# Autodesk Inventor assembly: Leg_Right
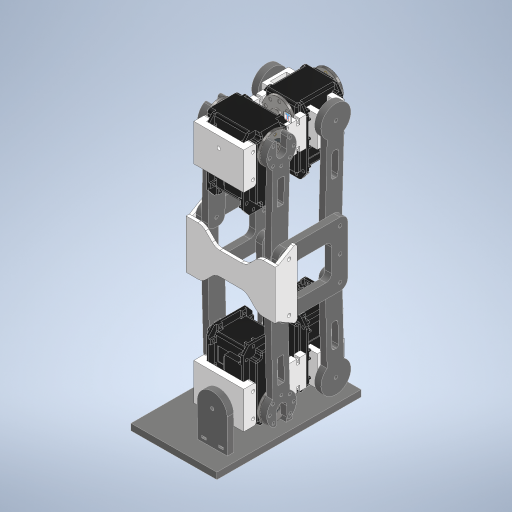
[picture p0: Inventor's stored thumbnail of the model, 512x512]
Saved by Autodesk Inventor 2024.3 (Build 283343000, 343)
## iProperties
Created: 2024-09-18
Part Number: Leg_Right
Document SubType Name: Assembly
Designer: 구지현
Author: 구지현
## Documents named in this file (20)
- C:\Users\구지현\Desktop\19th_intern_kdy_robot\부품\Lower_Body\Leg\Leg_Right.iam
- C:\Users\구지현\Documents\카카오톡 받은 파일\Hardware\ROBOTIS(Inventor 2024 ver.)\다이나믹셀\MX-64T+idle.ipt.iam
- C:\Users\구지현\Documents\카카오톡 받은 파일\Hardware\ROBOTIS(Inventor 2024 ver.)\다이나믹셀\MX-106T+idle.ipt.iam
- C:\Users\구지현\Documents\카카오톡 받은 파일\Hardware\ROBOTIS(Inventor 2024 ver.)\혼\64-106Horn.ipt
- C:\Users\구지현\Desktop\19th_intern_kdy_robot\부품\Lower_Body\Leg\Back_Ankle.ipt
- C:\Users\구지현\Desktop\19th_intern_kdy_robot\부품\Lower_Body\Leg\Foot_MIR.ipt
- C:\Users\구지현\Desktop\19th_intern_kdy_robot\부품\Lower_Body\Leg\Front_Ankle.ipt
- C:\Users\구지현\Desktop\19th_intern_kdy_robot\부품\Lower_Body\Leg\Knee.ipt
- C:\Users\구지현\Desktop\19th_intern_kdy_robot\부품\Lower_Body\Leg\Knee_Covers.ipt
- C:\Users\구지현\Desktop\19th_intern_kdy_robot\부품\Lower_Body\Leg\Leg_Connection_Parts_Back.ipt
- C:\Users\구지현\Desktop\19th_intern_kdy_robot\부품\Lower_Body\Leg\Leg_Connection_Parts_Front.ipt
- C:\Users\구지현\Desktop\19th_intern_kdy_robot\부품\Lower_Body\Leg\Leg_Foot_Connection_Parts.ipt
- C:\Users\구지현\Desktop\19th_intern_kdy_robot\부품\Lower_Body\Leg\Link_Fixation_Connector.ipt
- C:\Users\구지현\Desktop\19th_intern_kdy_robot\부품\Lower_Body\Leg\Link_Fixation_Connector_MIR.ipt
- Link_Fixation_Connector_left_left.ipt
- C:\Users\구지현\Desktop\19th_intern_kdy_robot\부품\Lower_Body\Leg\Link_Fixation_Connector_MIR_MIR.ipt
- C:\Users\구지현\Desktop\19th_intern_kdy_robot\부품\Lower_Body\Leg\Link_Fixation_Connector_MIR1.ipt
- C:\Users\구지현\Desktop\19th_intern_kdy_robot\부품\Lower_Body\Leg\Vertical_Fixation_Set.iam
- MX-106T+idle.ipt
- MX-64T+idle.ipt
## Components (32 placed, 16 different names)
1. MX-106T+idle.ipt:3 [sub-assembly] — 플러쉬:9, 각도:4, 플러쉬:10, 메이트:24, 메이트:25, 삽입:26, 삽입:27, 삽입:28, 삽입:29, 메이트:34, 메이트:35, 메이트:36
2. 64-106Horn:5 — 메이트:22, 메이트:23
3. MX-106T+idle.ipt:4 [sub-assembly] — 메이트:1, 메이트:2, 메이트:3, 메이트:6, 메이트:7, 메이트:8, 메이트:10, 메이트:11, 플러쉬:9, 각도:4, 플러쉬:10
4. 64-106Horn:6 — 메이트:12, 메이트:13
5. MX-64T+idle.ipt:3 [sub-assembly] — 플러쉬:13, 플러쉬:14, 삽입:30, 삽입:31, 삽입:32, 삽입:33, 삽입:34, 메이트:26, 메이트:27, 메이트:28, 메이트:30, 메이트:31, 메이트:32
6. 64-106Horn:7
7. MX-64T+idle.ipt:4 [sub-assembly] — 삽입:12, 메이트:9, 메이트:14, 메이트:15, 메이트:16, 메이트:18, 메이트:19, 메이트:20, 플러쉬:13, 플러쉬:14
8. 64-106Horn:8 — 삽입:10
9. Back_Ankle:1 — 삽입:10, 플러쉬:1, 각도:1, 삽입:14
10. Foot_MIR:1 — 삽입:13, 삽입:14
11. Front_Ankle:1 — 삽입:11, 플러쉬:1, 각도:1, 삽입:13
12. Knee:1 — 삽입:15, 삽입:18, 플러쉬:6, 플러쉬:7, 삽입:20, 삽입:21, 삽입:25, 삽입:36
13. Knee_Covers:1 — 삽입:20, 삽입:21, 삽입:22, 삽입:23
14. Leg_Connection_Parts_Front:1 — 메이트:12, 메이트:13, 플러쉬:2, 플러쉬:3, 삽입:15, 플러쉬:4, 각도:2
15. Leg_Foot_Connection_Parts:1 — 메이트:6, 메이트:7, 메이트:8, 삽입:11, 플러쉬:18
16. Link_Fixation_Connector_left_left:1 — 메이트:14, 메이트:15, 메이트:16, 메이트:17
17. Vertical_Fixation_Set:1 [sub-assembly] — 메이트:1, 메이트:2, 메이트:3, 삽입:12, 메이트:9
18. Leg_Connection_Parts_Front:2 — 메이트:10, 메이트:11, 플러쉬:2, 플러쉬:3, 삽입:17, 플러쉬:5, 각도:3
19. Link_Fixation_Connector_MIR1:2
20. Leg_Connection_Parts_Back:4 — 플러쉬:4, 각도:2, 삽입:18, 플러쉬:8, 메이트:21
21. Leg_Connection_Parts_Back:5 — 플러쉬:5, 각도:3, 삽입:19, 플러쉬:8, 메이트:17
22. Knee:2 — 삽입:17, 플러쉬:6, 플러쉬:7, 삽입:19, 삽입:22, 삽입:23, 삽입:24, 삽입:35
23. Link_Fixation_Connector:2 — 메이트:18, 메이트:19, 메이트:20, 메이트:21
24. Link_Fixation_Connector_MIR1:4 — 메이트:26, 메이트:27, 메이트:28, 메이트:29
25. Link_Fixation_Connector:3
26. Leg_Connection_Parts_Front:3 — 메이트:24, 메이트:25, 플러쉬:11, 플러쉬:12, 삽입:24, 플러쉬:15, 각도:5
27. Leg_Connection_Parts_Front:4 — 메이트:22, 메이트:23, 플러쉬:11, 플러쉬:12, 삽입:25, 플러쉬:16, 각도:6
28. Leg_Connection_Parts_Back:6 — 삽입:36, 플러쉬:16, 플러쉬:17, 각도:6, 메이트:29
29. Leg_Connection_Parts_Back:7 — 삽입:35, 플러쉬:15, 각도:5, 플러쉬:17, 메이트:33
30. Vertical_Fixation_Set:2 [sub-assembly] — 삽입:26, 삽입:27, 삽입:28, 삽입:29, 삽입:30, 삽입:31, 삽입:32, 삽입:33, 삽입:34
31. Link_Fixation_Connector_MIR_MIR:2 — 메이트:30, 메이트:31, 메이트:32, 메이트:33
32. Leg_Foot_Connection_Parts:3 — 메이트:34, 메이트:35, 메이트:36, 플러쉬:18
## Relationships (88: Mate 34, Insert 30, Flush 18, Angle 6)
- [Insert]: MX-106T+idle.ipt:3 ↔ 64-106Horn:5
- [Insert]: MX-106T+idle.ipt:4 ↔ 64-106Horn:6
- [Insert]: MX-64T+idle.ipt:3 ↔ 64-106Horn:7
- [Insert]: MX-64T+idle.ipt:4 ↔ 64-106Horn:8
- 메이트:1 [Mate] (0.1 mm): MX-106T+idle.ipt:4 ↔ Vertical_Fixation_Set:1
- 메이트:2 [Mate]: MX-106T+idle.ipt:4 ↔ Vertical_Fixation_Set:1
- 메이트:3 [Mate]: MX-106T+idle.ipt:4 ↔ Vertical_Fixation_Set:1
- 삽입:10 [Insert]: 64-106Horn:8 ↔ Back_Ankle:1
- 메이트:6 [Mate]: MX-106T+idle.ipt:4 ↔ Leg_Foot_Connection_Parts:1
- 메이트:7 [Mate] (0.1 mm): MX-106T+idle.ipt:4 ↔ Leg_Foot_Connection_Parts:1
- 메이트:8 [Mate]: MX-106T+idle.ipt:4 ↔ Leg_Foot_Connection_Parts:1
- 삽입:11 [Insert]: Front_Ankle:1 ↔ Leg_Foot_Connection_Parts:1
- 삽입:12 [Insert]: MX-64T+idle.ipt:4 ↔ Vertical_Fixation_Set:1
- 메이트:9 [Mate]: MX-64T+idle.ipt:4 ↔ Vertical_Fixation_Set:1
- 플러쉬:1 [Flush]: Back_Ankle:1 ↔ Front_Ankle:1
- 각도:1 [Angle] (0 deg): Back_Ankle:1 ↔ Front_Ankle:1
- 삽입:13 [Insert]: Foot_MIR:1 ↔ Front_Ankle:1
- 삽입:14 [Insert]: Back_Ankle:1 ↔ Foot_MIR:1
- 메이트:10 [Mate]: MX-106T+idle.ipt:4 ↔ Leg_Connection_Parts_Front:2
- 메이트:11 [Mate]: MX-106T+idle.ipt:4 ↔ Leg_Connection_Parts_Front:2
- 메이트:12 [Mate]: 64-106Horn:6 ↔ Leg_Connection_Parts_Front:1
- 메이트:13 [Mate]: 64-106Horn:6 ↔ Leg_Connection_Parts_Front:1
- 플러쉬:2 [Flush]: Leg_Connection_Parts_Front:1 ↔ Leg_Connection_Parts_Front:2
- 플러쉬:3 [Flush]: Leg_Connection_Parts_Front:1 ↔ Leg_Connection_Parts_Front:2
- 삽입:15 [Insert]: Knee:1 ↔ Leg_Connection_Parts_Front:1
- 삽입:17 [Insert]: Leg_Connection_Parts_Front:2 ↔ Knee:2
- 플러쉬:4 [Flush]: Leg_Connection_Parts_Front:1 ↔ Leg_Connection_Parts_Back:4
- 각도:2 [Angle] (0 deg): Leg_Connection_Parts_Front:1 ↔ Leg_Connection_Parts_Back:4
- 삽입:18 [Insert]: Knee:1 ↔ Leg_Connection_Parts_Back:4
- 플러쉬:5 [Flush]: Leg_Connection_Parts_Front:2 ↔ Leg_Connection_Parts_Back:5
- 각도:3 [Angle] (0 deg): Leg_Connection_Parts_Front:2 ↔ Leg_Connection_Parts_Back:5
- 플러쉬:6 [Flush]: Knee:1 ↔ Knee:2
- 플러쉬:7 [Flush]: Knee:1 ↔ Knee:2
- 삽입:19 [Insert]: Leg_Connection_Parts_Back:5 ↔ Knee:2
- 플러쉬:8 [Flush]: Leg_Connection_Parts_Back:4 ↔ Leg_Connection_Parts_Back:5
- 메이트:14 [Mate] (0.1 mm): MX-64T+idle.ipt:4 ↔ Link_Fixation_Connector_left_left:1
- 메이트:15 [Mate]: MX-64T+idle.ipt:4 ↔ Link_Fixation_Connector_left_left:1
- 메이트:16 [Mate]: MX-64T+idle.ipt:4 ↔ Link_Fixation_Connector_left_left:1
- 메이트:17 [Mate]: Link_Fixation_Connector_left_left:1 ↔ Leg_Connection_Parts_Back:5
- 메이트:18 [Mate] (0.1 mm): MX-64T+idle.ipt:4 ↔ Link_Fixation_Connector:2
- 메이트:19 [Mate]: MX-64T+idle.ipt:4 ↔ Link_Fixation_Connector:2
- 메이트:20 [Mate]: MX-64T+idle.ipt:4 ↔ Link_Fixation_Connector:2
- 메이트:21 [Mate]: Leg_Connection_Parts_Back:4 ↔ Link_Fixation_Connector:2
- 삽입:20 [Insert]: Knee:1 ↔ Knee_Covers:1
- 삽입:21 [Insert]: Knee:1 ↔ Knee_Covers:1
- 삽입:22 [Insert]: Knee_Covers:1 ↔ Knee:2
- 삽입:23 [Insert]: Knee_Covers:1 ↔ Knee:2
- 플러쉬:9 [Flush]: MX-106T+idle.ipt:3 ↔ MX-106T+idle.ipt:4
- 각도:4 [Angle] (0 deg): MX-106T+idle.ipt:3 ↔ MX-106T+idle.ipt:4
- 플러쉬:10 [Flush]: MX-106T+idle.ipt:3 ↔ MX-106T+idle.ipt:4
- 메이트:22 [Mate]: 64-106Horn:5 ↔ Leg_Connection_Parts_Front:4
- 메이트:23 [Mate]: 64-106Horn:5 ↔ Leg_Connection_Parts_Front:4
- 메이트:24 [Mate]: MX-106T+idle.ipt:3 ↔ Leg_Connection_Parts_Front:3
- 메이트:25 [Mate]: MX-106T+idle.ipt:3 ↔ Leg_Connection_Parts_Front:3
- 플러쉬:11 [Flush]: Leg_Connection_Parts_Front:3 ↔ Leg_Connection_Parts_Front:4
- 플러쉬:12 [Flush]: Leg_Connection_Parts_Front:3 ↔ Leg_Connection_Parts_Front:4
- 삽입:24 [Insert]: Knee:2 ↔ Leg_Connection_Parts_Front:3
- 삽입:25 [Insert]: Knee:1 ↔ Leg_Connection_Parts_Front:4
- 삽입:26 [Insert] (0.1 mm): MX-106T+idle.ipt:3 ↔ Vertical_Fixation_Set:2
- 삽입:27 [Insert] (0.1 mm): MX-106T+idle.ipt:3 ↔ Vertical_Fixation_Set:2
- 삽입:28 [Insert] (0.1 mm): MX-106T+idle.ipt:3 ↔ Vertical_Fixation_Set:2
- 삽입:29 [Insert] (0.1 mm): MX-106T+idle.ipt:3 ↔ Vertical_Fixation_Set:2
- 플러쉬:13 [Flush]: MX-64T+idle.ipt:3 ↔ MX-64T+idle.ipt:4
- 플러쉬:14 [Flush]: MX-64T+idle.ipt:3 ↔ MX-64T+idle.ipt:4
- 삽입:30 [Insert]: MX-64T+idle.ipt:3 ↔ Vertical_Fixation_Set:2
- 삽입:31 [Insert]: MX-64T+idle.ipt:3 ↔ Vertical_Fixation_Set:2
- 삽입:32 [Insert]: MX-64T+idle.ipt:3 ↔ Vertical_Fixation_Set:2
- 삽입:33 [Insert]: MX-64T+idle.ipt:3 ↔ Vertical_Fixation_Set:2
- 삽입:34 [Insert]: MX-64T+idle.ipt:3 ↔ Vertical_Fixation_Set:2
- 삽입:35 [Insert]: Knee:2 ↔ Leg_Connection_Parts_Back:7
- 플러쉬:15 [Flush]: Leg_Connection_Parts_Front:3 ↔ Leg_Connection_Parts_Back:7
- 각도:5 [Angle] (0 deg): Leg_Connection_Parts_Front:3 ↔ Leg_Connection_Parts_Back:7
- 삽입:36 [Insert]: Knee:1 ↔ Leg_Connection_Parts_Back:6
- 플러쉬:16 [Flush]: Leg_Connection_Parts_Front:4 ↔ Leg_Connection_Parts_Back:6
- 플러쉬:17 [Flush]: Leg_Connection_Parts_Back:6 ↔ Leg_Connection_Parts_Back:7
- 각도:6 [Angle] (0 deg): Leg_Connection_Parts_Front:4 ↔ Leg_Connection_Parts_Back:6
- 메이트:26 [Mate] (0.1 mm): MX-64T+idle.ipt:3 ↔ Link_Fixation_Connector_MIR1:4
- 메이트:27 [Mate]: MX-64T+idle.ipt:3 ↔ Link_Fixation_Connector_MIR1:4
- 메이트:28 [Mate]: MX-64T+idle.ipt:3 ↔ Link_Fixation_Connector_MIR1:4
- 메이트:29 [Mate]: Link_Fixation_Connector_MIR1:4 ↔ Leg_Connection_Parts_Back:6
- 메이트:30 [Mate] (0.1 mm): MX-64T+idle.ipt:3 ↔ Link_Fixation_Connector_MIR_MIR:2
- 메이트:31 [Mate]: MX-64T+idle.ipt:3 ↔ Link_Fixation_Connector_MIR_MIR:2
- 메이트:32 [Mate]: MX-64T+idle.ipt:3 ↔ Link_Fixation_Connector_MIR_MIR:2
- 메이트:33 [Mate]: Leg_Connection_Parts_Back:7 ↔ Link_Fixation_Connector_MIR_MIR:2
- 메이트:34 [Mate] (0.1 mm): MX-106T+idle.ipt:3 ↔ Leg_Foot_Connection_Parts:3
- 메이트:35 [Mate]: MX-106T+idle.ipt:3 ↔ Leg_Foot_Connection_Parts:3
- 메이트:36 [Mate]: MX-106T+idle.ipt:3 ↔ Leg_Foot_Connection_Parts:3
- 플러쉬:18 [Flush]: Leg_Foot_Connection_Parts:1 ↔ Leg_Foot_Connection_Parts:3
## Named parameters: d7_d130 = 0 mm, d8_d0_d1 = 0 mm, d9_d118 = 0 mm, d10_d140 = 0 mm
